# Autodesk Inventor assembly: Frame 1647030135921
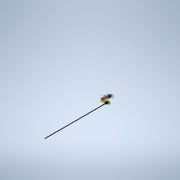
[picture p0: Inventor's stored thumbnail of the model, 180x180]
Saved by Autodesk Inventor 2022.2 (Build 262287000, 287)
## iProperties
_FrameDoc: Frame Assembly
_Version: 25.0.0
Created: 2022-03-11
Part Number: Frame 1647030135921
Document SubType Name: Assembly
Designer: foriw
Mass: 6846.58 g
Surface Area: 8196.39 cm^2
Volume: 2232.25 cm^3
Density: 3.06712 g/cm^3
Author: foriw
## Documents named in this file (30)
- H:\inventor ting\Mekatronik beercart git\Beercart CAD\Workspaces\Workspace\beercart assembly - mekatronik\Frame\Frame 1647030135921.iam
- H:\inventor ting\Mekatronik beercart git\Beercart CAD\Workspaces\Workspace\beercart assembly - mekatronik\Frame\Skeleton 1647030135922.ipt
- H:\inventor ting\Mekatronik beercart git\Beercart CAD\Workspaces\Workspace\beercart assembly - mekatronik\Frame\ISO 12633-2 20x20x2 1647030137505.ipt
- H:\inventor ting\Mekatronik beercart git\Beercart CAD\Workspaces\Workspace\beercart assembly - mekatronik\Frame\ISO 12633-2 20x20x2 1647030138110.ipt
- H:\inventor ting\Mekatronik beercart git\Beercart CAD\Workspaces\Workspace\beercart assembly - mekatronik\Frame\ISO 12633-2 20x20x2 1647030138225.ipt
- H:\inventor ting\Mekatronik beercart git\Beercart CAD\Workspaces\Workspace\beercart assembly - mekatronik\Frame\ISO 12633-2 20x20x2 1647030639616.ipt
- H:\inventor ting\Mekatronik beercart git\Beercart CAD\Workspaces\Workspace\beercart assembly - mekatronik\Frame\ISO 12633-2 20x20x2 1647030639707.ipt
- H:\inventor ting\Mekatronik beercart git\Beercart CAD\Workspaces\Workspace\beercart assembly - mekatronik\Frame\ISO 1035_2 10x 10 1647602096505.ipt
- H:\inventor ting\Mekatronik beercart git\Beercart CAD\Workspaces\Workspace\beercart assembly - mekatronik\Frame\ISO 1035_2 10x 10 1647602096566.ipt
- H:\inventor ting\Mekatronik beercart git\Beercart CAD\Workspaces\Workspace\beercart assembly - mekatronik\Frame\ISO 1035_2 10x 10 1647602096620.ipt
- H:\inventor ting\Mekatronik beercart git\Beercart CAD\Workspaces\Workspace\beercart assembly - mekatronik\Frame\ISO 12633-2 20x20x2 1647606177319.ipt
- H:\inventor ting\Mekatronik beercart git\Beercart CAD\Workspaces\Workspace\beercart assembly - mekatronik\Frame\ISO 12633-2 20x20x2 1647606177438.ipt
- H:\inventor ting\Mekatronik beercart git\Beercart CAD\Workspaces\Workspace\BackWheelMountingPlate.ipt
- H:\inventor ting\Mekatronik beercart git\Beercart CAD\Workspaces\Workspace\BackWheelMountingPlate_MIR_MIR.ipt
- H:\inventor ting\Mekatronik beercart git\Beercart CAD\Workspaces\Workspace\beercart assembly - mekatronik\Frame\ISO 1035_2 10x 10 1648211737860.ipt
- H:\inventor ting\Mekatronik beercart git\Beercart CAD\Workspaces\Workspace\bearing housing front.ipt
- H:\inventor ting\Mekatronik beercart git\Beercart CAD\Workspaces\Workspace\beercart assembly - mekatronik\Frame\ISO 12633-2 20x20x2 1648573909221.ipt
- H:\inventor ting\Mekatronik beercart git\Beercart CAD\Workspaces\Workspace\beercart assembly - mekatronik\Frame\ISO 12633-2 20x20x2 1648573975084.ipt
- H:\inventor ting\Mekatronik beercart git\Beercart CAD\Workspaces\Workspace\beercart assembly - mekatronik\Frame\ISO 12633-2 20x20x2 1648627088055.ipt
- H:\inventor ting\Mekatronik beercart git\Beercart CAD\Workspaces\Workspace\beercart assembly - mekatronik\Frame\ISO 12633-2 20x20x2 1648627088175.ipt
- H:\inventor ting\Mekatronik beercart git\Beercart CAD\Workspaces\Workspace\BackWheelMountingPlate_MIR4.ipt
- H:\inventor ting\Mekatronik beercart git\Beercart CAD\Workspaces\Workspace\beercart assembly - mekatronik\Frame\ISO 12633-2 20x20x2 1648631331581.ipt
- H:\inventor ting\Mekatronik beercart git\Beercart CAD\Workspaces\Workspace\beercart assembly - mekatronik\Frame\ISO 12633-2 20x20x2 1649085652950.ipt
- H:\inventor ting\Mekatronik beercart git\Beercart CAD\Workspaces\Workspace\beercart assembly - mekatronik\Frame\ISO 12633-2 20x20x2 1649085653040.ipt
- H:\inventor ting\Mekatronik beercart git\Beercart CAD\Workspaces\Workspace\backWheelNoMotor brake mount.ipt
- H:\inventor ting\Mekatronik beercart git\Beercart CAD\Workspaces\Workspace\beercart assembly - mekatronik\Frame\ISO 12633-2 20x20x2 1649154464355.ipt
- H:\inventor ting\Mekatronik beercart git\Beercart CAD\Workspaces\Workspace\BackWheelMotorMountSpacer.ipt
- H:\inventor ting\Mekatronik beercart git\Beercart CAD\Workspaces\Workspace\beercart assembly - mekatronik\Frame\FrontWheelFrameNew.iam
- H:\inventor ting\Mekatronik beercart git\Beercart CAD\Workspaces\Workspace\beercart assembly - mekatronik\Frame\ISO 12633-2 20x20x2 1649415836960.ipt
- H:\inventor ting\Mekatronik beercart git\Beercart CAD\Workspaces\Workspace\headset bearing.ipt
## Components (29 placed, 23 different names)
1. bearing housing front:1 — Mate:14, Insert:4
2. Reference Skeleton
3. ISO 12633-2 20x20x2 - 329,99:2
4. ISO 12633-2 20x20x2 - 290:1
5. ISO 12633-2 20x20x2 - 162,48:3
6. ISO 12633-2 20x20x2 - 250,13:1
7. ISO 12633-2 20x20x2 - 250,13:2
8. ISO 1035/2 10x 10 - 79,02:1 — Mate:14
9. ISO 1035/2 10x 10 - 64,59:1
10. ISO 1035/2 10x 10 - 64,59:2
11. ISO 12633-2 20x20x2 - 123,73:1 — Mate:1, Mate:3
12. ISO 12633-2 20x20x2 - 123,73:2 — Mate:2, Mate:4, Mate:5
13. BackWheelMountingPlate:1 — Flush:6, Rotational:2, Rigid:1
14. BackWheelMountingPlate_MIR_MIR:1
15. ISO 1035/2 10x 10 - 79,02:1
16. ISO 12633-2 20x20x2 - 360,44:1
17. ISO 12633-2 20x20x2 - 105,43:1 — Flush:6, Rotational:2, Rigid:1
18. ISO 12633-2 20x20x2 - 107,97:1 — Flush:9, Flush:11, Flush:12, Flush:13, Rigid:2
19. ISO 12633-2 20x20x2 - 110,27:1
20. BackWheelMountingPlate_MIR4:1 — Flush:9, Rigid:2
21. ISO 12633-2 20x20x2 - 360,44:1
22. ISO 12633-2 20x20x2 - 113,16:1 — Flush:14
23. ISO 12633-2 20x20x2 - 113,2:1 — Flush:10
24. backWheelNoMotor brake mount:1 — Flush:10, Flush:14
25. ISO 12633-2 20x20x2 - 105,43:1
26. BackWheelMotorMountSpacer:1 — Flush:11, Flush:12, Flush:13
27. FrontWheelFrameNew:1 [sub-assembly] — Insert:3, Insert:4
28. headset bearing:1 — Insert:3
29. ISO 12633-2 20x20x2 - 51,61:1
## Relationships (19: Flush 8, Mate 6, WeldJoint 2, Insert 2, RevoluteJoint 1)
- Mate:1: ISO 12633-2 20x20x2 - 123,73:1
- Mate:2: ISO 12633-2 20x20x2 - 123,73:2
- Mate:3: ISO 12633-2 20x20x2 - 123,73:1
- Mate:4: ISO 12633-2 20x20x2 - 123,73:2
- Mate:5: ISO 12633-2 20x20x2 - 123,73:2
- Mate:14: bearing housing front:1 ↔ ISO 1035/2 10x 10 - 79,02:1
- [Flush]: bearing housing front:1 ↔ ISO 1035/2 10x 10 - 79,02:1
- Flush:6: BackWheelMountingPlate:1 ↔ ISO 12633-2 20x20x2 - 105,43:1
- Rotational:2 [RevoluteJoint]: BackWheelMountingPlate:1 ↔ ISO 12633-2 20x20x2 - 105,43:1
- Flush:9: ISO 12633-2 20x20x2 - 107,97:1 ↔ BackWheelMountingPlate_MIR4:1
- Flush:10: ISO 12633-2 20x20x2 - 113,2:1 ↔ backWheelNoMotor brake mount:1
- Rigid:1 [WeldJoint]: BackWheelMountingPlate:1 ↔ ISO 12633-2 20x20x2 - 105,43:1
- Flush:11: ISO 12633-2 20x20x2 - 107,97:1 ↔ BackWheelMotorMountSpacer:1
- Flush:12: ISO 12633-2 20x20x2 - 107,97:1 ↔ BackWheelMotorMountSpacer:1
- Flush:13: ISO 12633-2 20x20x2 - 107,97:1 ↔ BackWheelMotorMountSpacer:1
- Flush:14: ISO 12633-2 20x20x2 - 113,16:1 ↔ backWheelNoMotor brake mount:1
- Insert:3: FrontWheelFrameNew:1 ↔ headset bearing:1
- Insert:4 (1 mm): bearing housing front:1 ↔ FrontWheelFrameNew:1
- Rigid:2 [WeldJoint]: ISO 12633-2 20x20x2 - 107,97:1 ↔ BackWheelMountingPlate_MIR4:1
## Named parameters: d22_d2 = 0 mm, d23_d3 = 0 mm
